# Autodesk Inventor assembly: leg_ass_1_MIR
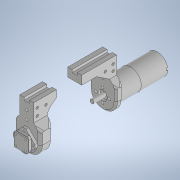
[picture p0: Inventor's stored thumbnail of the model, 180x180]
Saved by Autodesk Inventor 2020 (Build 240168000, 168)
## iProperties
Created: 2019-05-04
Part Number: leg_ass_1_MIR
Document SubType Name: Assembly
Designer: psrob
Author: psrob
## Documents named in this file (5)
- E:\projects-2\project dog gen2\hardware\leg_ass_1_MIR.iam
- E:\projects-2\project dog gen2\hardware\dog_bone_1_MIR.ipt
- E:\projects-2\project dog gen2\hardware\motor_2_MIR.ipt
- E:\projects-2\project dog gen2\hardware\dog_bone_3_MIR1.ipt
- E:\projects-2\project dog gen2\hardware\encoder_ass_MIR.iam
## Components (4 placed, 4 different names)
1. dog_bone_1_MIR:1 — Angle:1, Flush:1, Insert:8, Insert:9
2. motor_2_MIR:1 — Mate:1
3. dog_bone_3_MIR1:1 — Angle:1, Mate:1, Flush:1
4. encoder_ass_MIR:1 [sub-assembly] — Insert:8, Insert:9
## Relationships (5: Insert 2, Angle 1, Mate 1, Flush 1)
- Angle:1 (0 deg): dog_bone_1_MIR:1 ↔ dog_bone_3_MIR1:1
- Mate:1: motor_2_MIR:1 ↔ dog_bone_3_MIR1:1
- Flush:1: dog_bone_1_MIR:1 ↔ dog_bone_3_MIR1:1
- Insert:8: dog_bone_1_MIR:1 ↔ encoder_ass_MIR:1
- Insert:9: dog_bone_1_MIR:1 ↔ encoder_ass_MIR:1
